# Autodesk Inventor assembly: StorageAssembly-ver6-1111-2021
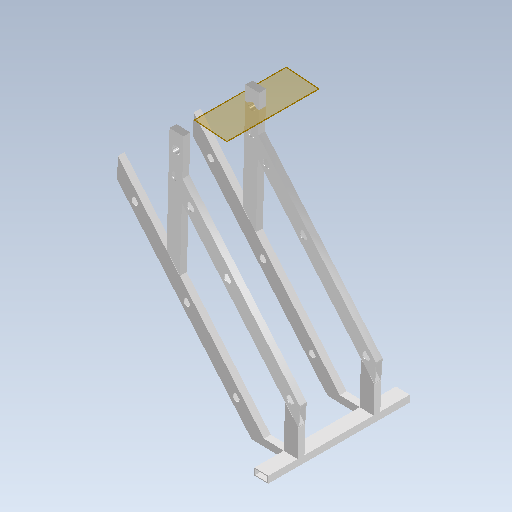
[picture p0: Inventor's stored thumbnail of the model, 512x512]
Saved by Autodesk Inventor 2021 (Build 250183000, 183)
## iProperties
Created: 2021-03-11
Part Number: StorageAssembly-ver6-1111-2021
Document SubType Name: Assembly
Designer: CMurray
Author: CMurray
## Documents named in this file (6)
- C:\Users\CMurray\OneDrive\Documents\GitHub\RoboticsCad1111\PHRC CADD\2020 Infinite Recharge\Storage\Assemblies\StorageAssembly-ver6-1111-2021.iam
- C:\Users\CMurray\OneDrive\Documents\GitHub\RoboticsCad1111\PHRC CADD\2020 Infinite Recharge\Storage\Parts\AngleBrace.ver2-1111-2020.ipt
- C:\Users\CMurray\OneDrive\Documents\GitHub\RoboticsCad1111\PHRC CADD\2020 Infinite Recharge\Storage\Parts\IntakeBrace.ver1-1111-2020.ipt
- C:\Users\CMurray\OneDrive\Documents\GitHub\RoboticsCad1111\PHRC CADD\2020 Infinite Recharge\Shooting\Parts\SmallAnglesSupport.ver1-1111-2020_MIR.ipt
- C:\Users\CMurray\OneDrive\Documents\GitHub\RoboticsCad1111\PHRC CADD\2020 Infinite Recharge\Storage\Assemblies\StorageAssembly.ver3-1111-2020.iam
- C:\Users\CMurray\OneDrive\Documents\GitHub\RoboticsCad1111\PHRC CADD\2020 Infinite Recharge\Storage\Parts\StorageSupport.ver2-1111-2021.ipt
## Components (8 placed, 5 different names)
1. IntakeBrace.ver1-1111-2020:1 — Mate:1, Flush:1, Mate:2, Flush:2, Flush:4, Flush:5, Mate:7, Flush:7, Flush:8
2. SmallAnglesSupport.ver1-1111-2020_MIR:1 — Mate:1, Flush:1, Mate:3, Flush:3, Flush:4, Mate:4
3. SmallAnglesSupport.ver1-1111-2020_MIR:2 — Mate:2, Flush:2, Flush:5, Mate:5, Flush:6, Mate:6
4. AngleBrace.ver2-1111-2020:1 — Mate:3, Flush:3, Mate:4, Mate:15
5. AngleBrace.ver2-1111-2020:2 — Mate:5, Flush:6, Mate:6, Flush:13, Mate:16
6. StorageAssembly.ver3-1111-2020:1 [sub-assembly] — Mate:7, Flush:7, Flush:8, Flush:12, Mate:13, Mate:14
7. StorageSupport.ver2-1111-2021:1 — Flush:12, Mate:13, Mate:15
8. StorageSupport.ver2-1111-2021:2 — Flush:13, Mate:14, Mate:16
## Relationships (22: Mate 11, Flush 11)
- Mate:1: IntakeBrace.ver1-1111-2020:1 ↔ SmallAnglesSupport.ver1-1111-2020_MIR:1
- Flush:1: IntakeBrace.ver1-1111-2020:1 ↔ SmallAnglesSupport.ver1-1111-2020_MIR:1
- Mate:2: IntakeBrace.ver1-1111-2020:1 ↔ SmallAnglesSupport.ver1-1111-2020_MIR:2
- Flush:2: IntakeBrace.ver1-1111-2020:1 ↔ SmallAnglesSupport.ver1-1111-2020_MIR:2
- Mate:3: SmallAnglesSupport.ver1-1111-2020_MIR:1 ↔ AngleBrace.ver2-1111-2020:1
- Flush:3: SmallAnglesSupport.ver1-1111-2020_MIR:1 ↔ AngleBrace.ver2-1111-2020:1
- Flush:4 (107.95 mm): IntakeBrace.ver1-1111-2020:1 ↔ SmallAnglesSupport.ver1-1111-2020_MIR:1
- Flush:5 (107.95 mm): IntakeBrace.ver1-1111-2020:1 ↔ SmallAnglesSupport.ver1-1111-2020_MIR:2
- Mate:4: SmallAnglesSupport.ver1-1111-2020_MIR:1 ↔ AngleBrace.ver2-1111-2020:1
- Mate:5: SmallAnglesSupport.ver1-1111-2020_MIR:2 ↔ AngleBrace.ver2-1111-2020:2
- Flush:6: SmallAnglesSupport.ver1-1111-2020_MIR:2 ↔ AngleBrace.ver2-1111-2020:2
- Mate:6: SmallAnglesSupport.ver1-1111-2020_MIR:2 ↔ AngleBrace.ver2-1111-2020:2
- Mate:7: IntakeBrace.ver1-1111-2020:1 ↔ StorageAssembly.ver3-1111-2020:1
- Flush:7 (107.95 mm): IntakeBrace.ver1-1111-2020:1 ↔ StorageAssembly.ver3-1111-2020:1
- Flush:8: IntakeBrace.ver1-1111-2020:1 ↔ StorageAssembly.ver3-1111-2020:1
- Flush:11 (-1.016 mm)
- Flush:12: StorageAssembly.ver3-1111-2020:1 ↔ StorageSupport.ver2-1111-2021:1
- Mate:13: StorageAssembly.ver3-1111-2020:1 ↔ StorageSupport.ver2-1111-2021:1
- Flush:13: AngleBrace.ver2-1111-2020:2 ↔ StorageSupport.ver2-1111-2021:2
- Mate:14: StorageAssembly.ver3-1111-2020:1 ↔ StorageSupport.ver2-1111-2021:2
- Mate:15: AngleBrace.ver2-1111-2020:1 ↔ StorageSupport.ver2-1111-2021:1
- Mate:16: AngleBrace.ver2-1111-2020:2 ↔ StorageSupport.ver2-1111-2021:2
